# Autodesk Inventor assembly: ASY MSC 900.2 support
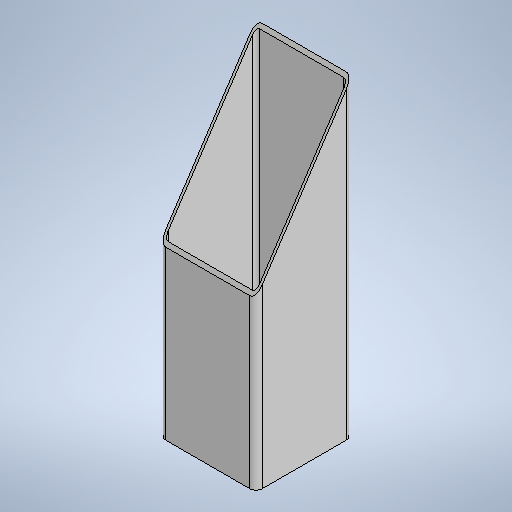
[picture p0: Inventor's stored thumbnail of the model, 512x512]
Saved by Autodesk Inventor 2025 (Build 290162010, 162A)
## iProperties
Created: 2024-08-15
Part Number: ASY MSC 900.2 support
Document SubType Name: Assembly
Designer: admin
Stock Number: МОО 900.2 опора
Author: admin
Revision Number: 8
## Documents named in this file (5)
- C:\Users\admin\YandexDisk-badmisterfox\домашниий пк\Inventor\Manturovo\Manturovo_Se-clar\ASY MSC 900.2 support.iam
- C:\Users\admin\YandexDisk-badmisterfox\домашниий пк\Inventor\Manturovo\Manturovo_Se-clar\MSC 903 base tube.ipt
- C:\Users\admin\YandexDisk-badmisterfox\домашниий пк\Inventor\Manturovo\Manturovo_Se-clar\MSC 904 flange base tube.ipt
- C:\Users\admin\YandexDisk-badmisterfox\домашниий пк\Inventor\Manturovo\Manturovo_Se-clar\MSC 905 flange base tube support.ipt
- C:\Users\admin\YandexDisk-badmisterfox\домашниий пк\Inventor\Manturovo\Manturovo_Se-clar\MSC 908 tube support 3.ipt
## Components (4 placed, 4 different names)
1. MSC 903 base tube.ipt:1 — Rotational:2
2. MSC 904 flange base tube.ipt:1 — Rotational:2
3. MSC 905 flange base tube support.ipt:1 — Rigid:3
4. MSC 908 tube support 3.ipt:1 — Rigid:3
## Relationships (3: WeldJoint 2, RevoluteJoint 1)
- Rotational:2 [RevoluteJoint]: MSC 903 base tube.ipt:1 ↔ MSC 904 flange base tube.ipt:1
- [WeldJoint]: MSC 903 base tube.ipt:1 ↔ MSC 905 flange base tube support.ipt:1
- Rigid:3 [WeldJoint]: MSC 905 flange base tube support.ipt:1 ↔ MSC 908 tube support 3.ipt:1
